# Autodesk Inventor assembly: 1_Base
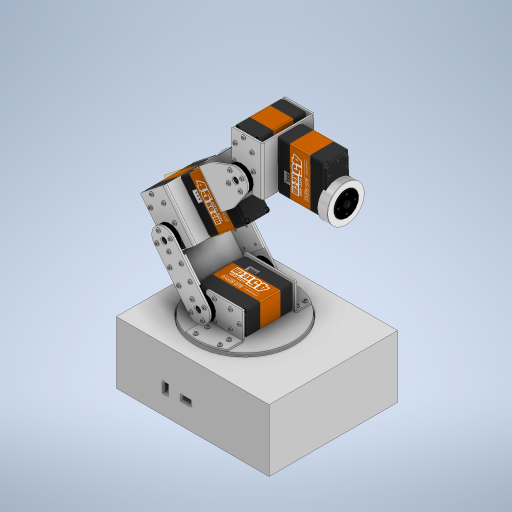
[picture p0: Inventor's stored thumbnail of the model, 512x512]
Saved by Autodesk Inventor 2024.2 (Build 282272000, 272)
## iProperties
Created: 2023-08-24
Part Number: 1_Base
Document SubType Name: Assembly
Designer: chanh
Author: chanh
## Documents named in this file (32)
- C:\Users\chanh\내 드라이브\로봇\Humanoid\Roboin Humanoid Project\Inventor\rh_plus_7_axis_robot_arm_hardware\Assembly\2_Arm.iam
- C:\Users\chanh\내 드라이브\로봇\Humanoid\Roboin Humanoid Project\Inventor\rh_plus_7_axis_robot_arm_hardware\Part\HTD-45H, Horn\HTD-45H\HTD-45H.ipt
- C:\Users\chanh\내 드라이브\로봇\Humanoid\Roboin Humanoid Project\Inventor\rh_plus_7_axis_robot_arm_hardware\Part\Frame\axis_1_top_frame.ipt
- C:\Users\chanh\내 드라이브\로봇\Humanoid\Roboin Humanoid Project\Inventor\rh_plus_7_axis_robot_arm_hardware\Part\Other Parts\Aluminum_Profile_4040_100.14mm_top.ipt
- C:\Users\chanh\내 드라이브\로봇\Humanoid\Roboin Humanoid Project\Inventor\rh_plus_7_axis_robot_arm_hardware\Part\Other Parts\Aluminum_Profile_4040_40.10mm_right.ipt
- C:\Users\chanh\내 드라이브\로봇\Humanoid\Roboin Humanoid Project\Inventor\rh_plus_7_axis_robot_arm_hardware\Part\Other Parts\Aluminum_Profile_4040_40.10mm_left.ipt
- C:\Users\chanh\내 드라이브\로봇\Humanoid\Roboin Humanoid Project\Inventor\rh_plus_7_axis_robot_arm_hardware\Part\Other Parts\Aluminum_Profile_4040_100.14mm_bottom.ipt
- C:\Users\chanh\내 드라이브\로봇\Humanoid\Roboin Humanoid Project\Inventor\rh_plus_7_axis_robot_arm_hardware\Part\HTD-45H, Horn\HTD-45H\M2x32.ipt
- C:\Users\chanh\내 드라이브\로봇\Humanoid\Roboin Humanoid Project\Inventor\rh_plus_7_axis_robot_arm_hardware\Part\HTD-45H, Horn\Horn\Top Horn.ipt
- C:\Users\chanh\내 드라이브\로봇\Humanoid\Roboin Humanoid Project\Inventor\rh_plus_7_axis_robot_arm_hardware\Part\Bolt, Bearing, Nut, Washer\M2x6 Round Bolt.ipt
- C:\Users\chanh\내 드라이브\로봇\Humanoid\Roboin Humanoid Project\Inventor\rh_plus_7_axis_robot_arm_hardware\Part\Bolt, Bearing, Nut, Washer\M2x35 Round Bolt.ipt
- C:\Users\chanh\내 드라이브\로봇\Humanoid\Roboin Humanoid Project\Inventor\rh_plus_7_axis_robot_arm_hardware\Part\Frame\axis_2_bottom_frame.ipt
- C:\Users\chanh\내 드라이브\로봇\Humanoid\Roboin Humanoid Project\Inventor\rh_plus_7_axis_robot_arm_hardware\Part\Bolt, Bearing, Nut, Washer\AXK5070+AS Bearing.ipt
- C:\Users\chanh\내 드라이브\로봇\Humanoid\Roboin Humanoid Project\Inventor\rh_plus_7_axis_robot_arm_hardware\Part\Bolt, Bearing, Nut, Washer\M2x6 Bolt.ipt
- C:\Users\chanh\내 드라이브\로봇\Humanoid\Roboin Humanoid Project\Inventor\rh_plus_7_axis_robot_arm_hardware\Part\HTD-45H, Horn\HTD-45H\HTD-45H.iam
- C:\Users\chanh\내 드라이브\로봇\Humanoid\Roboin Humanoid Project\Inventor\rh_plus_7_axis_robot_arm_hardware\Part\HTD-45H, Horn\Horn\M3x6.ipt
- C:\Users\chanh\내 드라이브\로봇\Humanoid\Roboin Humanoid Project\Inventor\rh_plus_7_axis_robot_arm_hardware\Part\Frame\axis_2_bottom_L_frame(top).ipt
- C:\Users\chanh\내 드라이브\로봇\Humanoid\Roboin Humanoid Project\Inventor\rh_plus_7_axis_robot_arm_hardware\Part\Frame\axis_2_bottom_L_frame(bottom).ipt
- C:\Users\chanh\내 드라이브\로봇\Humanoid\Roboin Humanoid Project\Inventor\rh_plus_7_axis_robot_arm_hardware\Part\HTD-45H, Horn\Horn\Bottom Horn.ipt
- C:\Users\chanh\내 드라이브\로봇\Humanoid\Roboin Humanoid Project\Inventor\rh_plus_7_axis_robot_arm_hardware\Part\Bolt, Bearing, Nut, Washer\M2x4 Round Bolt.ipt
- C:\Users\chanh\내 드라이브\로봇\Humanoid\Roboin Humanoid Project\Inventor\rh_plus_7_axis_robot_arm_hardware\Part\Frame\axis_3_bottom_frame(top).ipt
- C:\Users\chanh\내 드라이브\로봇\Humanoid\Roboin Humanoid Project\Inventor\rh_plus_7_axis_robot_arm_hardware\Part\Frame\axis_3_bottom_frame(bottom).ipt
- C:\Users\chanh\내 드라이브\로봇\Humanoid\Roboin Humanoid Project\Inventor\rh_plus_7_axis_robot_arm_hardware\Part\Frame\axis_3_bottom_frame(middle).ipt
- C:\Users\chanh\내 드라이브\로봇\Humanoid\Roboin Humanoid Project\Inventor\rh_plus_7_axis_robot_arm_hardware\Part\Frame\axis_3_top_frame.ipt
- C:\Users\chanh\내 드라이브\로봇\Humanoid\Roboin Humanoid Project\Inventor\rh_plus_7_axis_robot_arm_hardware\Part\Frame\axis_4_top_frame.ipt
- C:\Users\chanh\내 드라이브\로봇\Humanoid\Roboin Humanoid Project\Inventor\rh_plus_7_axis_robot_arm_hardware\Part\Frame\axis_5_bottom_frame.ipt
- C:\Users\chanh\내 드라이브\로봇\Humanoid\Roboin Humanoid Project\Inventor\rh_plus_7_axis_robot_arm_hardware\Part\Frame\axis_5_top_frame.ipt
- C:\Users\chanh\내 드라이브\로봇\Humanoid\Roboin Humanoid Project\Inventor\rh_plus_7_axis_robot_arm_hardware\Part\Bolt, Bearing, Nut, Washer\2030 Teflon Sheet.ipt
- C:\Users\chanh\내 드라이브\로봇\Humanoid\Roboin Humanoid Project\Inventor\rh_plus_7_axis_robot_arm_hardware\Part\Frame\axis_6_top_frame.ipt
- C:\Users\chanh\내 드라이브\로봇\Humanoid\Roboin Humanoid Project\Inventor\rh_plus_7_axis_robot_arm_hardware\Part\HTD-45H, Horn\Horn\M3x5.ipt
- C:\Users\chanh\내 드라이브\로봇\Humanoid\Roboin Humanoid Project\Inventor\rh_plus_7_axis_robot_arm_hardware\Part\Other Parts\Bottom_Cover.ipt
- C:\Users\chanh\내 드라이브\로봇\Humanoid\Roboin Humanoid Project\Inventor\rh_plus_7_axis_robot_arm_hardware\Part\Bolt, Bearing, Nut, Washer\M5x14.ipt
## Components (161 placed, 30 different names)
1. Aluminum_Profile_4040_100.14mm_top:1 — Flush:13, Flush:14, Mate:2, Mate:3, Flush:15, Flush:16, Mate:4, Flush:17, Flush:18, Mate:6
2. Aluminum_Profile_4040_40.10mm_right:1 — Mate:3, Flush:15, Flush:16
3. Aluminum_Profile_4040_40.10mm_left:1 — Mate:4, Flush:17, Flush:18, Mate:5, Flush:20
4. Aluminum_Profile_4040_100.14mm_bottom:1 — Flush:19, Mate:5, Flush:20, Mate:19, Flush:27
5. Bottom_Cover:1 — Mate:19, Mate:20, Flush:27
6. HTD-45H:1 — Rotational:1, Mate:1, Flush:1, Flush:2, Flush:12, Flush:13, Flush:14, Mate:2, Flush:19, Rigid:1, Rigid:2, Mate:7, Mate:8
7. axis_1_top_frame:1 — Flush:11, Flush:12, Mate:6, Mate:9, Mate:20, Rigid:160, Rigid:161, Rigid:162, Rigid:163, Rigid:164, Rigid:165, Rigid:166, Rigid:167, Rigid:168, Rigid:169, Rigid:170
8. HTD-45H:2 [sub-assembly] — Flush:21, Mate:11, Flush:23, Flush:24, Mate:13, Mate:17, Rotational:2, Rigid:114
9. axis_2_bottom_frame:1 — Rigid:10, Rigid:18, Rigid:19, Rigid:20, Rigid:21, Flush:21, Mate:11, Mate:14
10. axis_2_bottom_L_frame(top):1 — Flush:23, Flush:24, Mate:13, Mate:14, Rigid:23, Rigid:24, Rigid:25, Rigid:26, Rigid:27, Rigid:28, Rigid:29, Rigid:30, Rigid:31
11. axis_2_bottom_L_frame(bottom):1 — Mate:17, Rigid:32, Rigid:33, Rigid:34, Rigid:35, Rigid:36, Rigid:37, Rigid:38, Rigid:39, Rigid:40, Rigid:41, Rigid:42, Rigid:43
12. HTD-45H:3 [sub-assembly] — Rotational:3, Flush:25, Mate:18, Flush:26
13. axis_3_bottom_frame(top):1 — Rigid:44, Rigid:45, Rigid:48, Rigid:49, Rigid:50, Rigid:51, Rigid:52, Rigid:53, Rigid:54, Rigid:55, Rigid:56, Rigid:57, Rigid:58, Rigid:59, Rigid:60
14. axis_3_bottom_frame(middle):1 — Rigid:48, Rigid:104
15. axis_3_bottom_frame(bottom):1 — Rigid:61, Rigid:62, Rigid:63, Rigid:64, Rigid:65, Rigid:66, Rigid:67, Rigid:68, Rigid:69, Rigid:70, Rigid:71, Rigid:72, Rigid:102, Rigid:103, Rigid:104
16. axis_3_top_frame:1 — Flush:25, Mate:18, Flush:26, Rigid:74, Rigid:75, Rigid:76, Rigid:77, Rigid:78, Rigid:79, Rigid:80, Rigid:81, Rigid:82, Rigid:83, Rigid:84, Rigid:85, Rigid:86, Rigid:87, Rigid:88, Rigid:89, Rigid:90
17. HTD-45H:4 — Rigid:90, Rigid:91, Rigid:92, Rotational:4, Rigid:106
18. 2030 Teflon Sheet:1 — Rigid:107
19. axis_4_top_frame:1 — Rigid:106, Rigid:107, Rigid:155, Rigid:156, Rigid:157, Rigid:158
20. HTD-45H:5 [sub-assembly] — Rigid:105, Rotational:5
21. 2030 Teflon Sheet:2 — Rigid:108
22. axis_5_bottom_frame:1 — Rigid:99, Rigid:108, Rigid:126, Rigid:127, Rigid:128, Rigid:129, Rigid:130, Rigid:131, Rigid:132, Rigid:133, Rigid:134, Rigid:135, Rigid:136, Rigid:137, Rigid:138, Rigid:159
23. axis_5_top_frame:1 — Rigid:105, Rigid:111, Rigid:139, Rigid:140, Rigid:141, Rigid:142, Rigid:143, Rigid:144, Rigid:145, Rigid:146, Rigid:147, Rigid:148, Rigid:149, Rigid:150, Rigid:151, Rigid:152, Rigid:153, Rigid:154
24. HTD-45H:6 — Rigid:111, Rigid:112, Rotational:6
25. 2030 Teflon Sheet:3 — Rigid:125
26. axis_6_top_frame:1 — Rigid:112, Rigid:120, Rigid:121, Rigid:122, Rigid:123, Rigid:125
27. M2x32:1 — Rigid:2
28. M2x32:2 — Rigid:1
29. Top Horn:1 — Rotational:1, Rigid:10, Rigid:22
30. M5x14:1 — Rigid:160
31. M5x14:2 — Rigid:163
32. M5x14:3 — Rigid:161
33. M5x14:4 — Rigid:162
34. M3x6:1 — Rigid:22
35. M2x6 Round Bolt:3 — Rigid:168
36. M2x6 Round Bolt:4 — Rigid:170
37. M2x6 Round Bolt:5 — Rigid:169
38. AXK5070+AS Bearing:1 — Mate:7, Mate:8, Mate:9
39. M2x6 Round Bolt:1 — Rigid:167
40. M2x6 Round Bolt:2 — Rigid:166
41. M2x35 Round Bolt:1 — Rigid:165
42. M2x35 Round Bolt:2 — Rigid:164
43. Bottom Horn:5 — Rigid:102
44. Top Horn:2 — Rotational:2, Rigid:44, Rigid:113
45. M3x5:1 — Rigid:114
46. M3x6:2 — Rigid:113
47. M2x6 Bolt:1 — Rigid:18
48. M2x6 Bolt:2 — Rigid:19
49. M2x6 Bolt:3 — Rigid:20
50. M2x6 Bolt:4 — Rigid:21
51. M2x4 Round Bolt:1 — Rigid:23
52. M2x4 Round Bolt:2 — Rigid:24
53. M2x4 Round Bolt:3 — Rigid:25
54. M2x4 Round Bolt:4 — Rigid:26
55. M2x4 Round Bolt:5 — Rigid:27
56. M2x4 Round Bolt:6 — Rigid:28
57. M2x4 Round Bolt:7 — Rigid:29
58. M2x4 Round Bolt:8 — Rigid:30
59. M2x4 Round Bolt:9 — Rigid:31
60. M2x4 Round Bolt:10 — Rigid:32
61. M2x4 Round Bolt:11 — Rigid:33
62. M2x4 Round Bolt:12 — Rigid:34
63. M2x4 Round Bolt:13 — Rigid:35
64. M2x4 Round Bolt:14 — Rigid:36
65. M2x4 Round Bolt:15 — Rigid:37
66. M2x4 Round Bolt:16 — Rigid:38
67. M2x4 Round Bolt:17 — Rigid:39
68. M2x4 Round Bolt:18 — Rigid:40
69. M2x4 Round Bolt:19 — Rigid:41
70. M2x4 Round Bolt:20 — Rigid:42
71. M2x4 Round Bolt:21 — Rigid:43
72. Bottom Horn:4 — Rigid:103, Rigid:116
73. Top Horn:3 — Rotational:3, Rigid:45, Rigid:115
74. M3x5:2 — Rigid:116
75. M3x6:3 — Rigid:115
76. M2x4 Round Bolt:22 — Rigid:50
77. M2x4 Round Bolt:23 — Rigid:51
78. M2x4 Round Bolt:24 — Rigid:52
79. M2x4 Round Bolt:25 — Rigid:49
80. M2x4 Round Bolt:26 — Rigid:53
81. M2x4 Round Bolt:27 — Rigid:54
82. M2x4 Round Bolt:28 — Rigid:55
83. M2x4 Round Bolt:29 — Rigid:56
84. M2x4 Round Bolt:30 — Rigid:57
85. M2x4 Round Bolt:31 — Rigid:58
86. M2x4 Round Bolt:32 — Rigid:59
87. M2x4 Round Bolt:33 — Rigid:60
88. M2x4 Round Bolt:34 — Rigid:61
89. M2x4 Round Bolt:35 — Rigid:62
90. M2x4 Round Bolt:36 — Rigid:63
91. M2x4 Round Bolt:37 — Rigid:64
92. M2x4 Round Bolt:38 — Rigid:65
93. M2x4 Round Bolt:39 — Rigid:66
94. M2x4 Round Bolt:40 — Rigid:67
95. M2x4 Round Bolt:41 — Rigid:68
96. M2x4 Round Bolt:42 — Rigid:69
97. M2x4 Round Bolt:43 — Rigid:70
98. M2x4 Round Bolt:44 — Rigid:71
99. M2x4 Round Bolt:45 — Rigid:72
100. M2x4 Round Bolt:46 — Rigid:74
101. M2x4 Round Bolt:47 — Rigid:75
102. M2x4 Round Bolt:48 — Rigid:76
103. M2x4 Round Bolt:49 — Rigid:77
104. M2x4 Round Bolt:50 — Rigid:78
105. M2x4 Round Bolt:51 — Rigid:79
106. M2x4 Round Bolt:52 — Rigid:80
107. M2x4 Round Bolt:53 — Rigid:81
108. M2x4 Round Bolt:54 — Rigid:82
109. M2x4 Round Bolt:55 — Rigid:83
110. M2x4 Round Bolt:56 — Rigid:84
111. M2x4 Round Bolt:57 — Rigid:85
112. M2x4 Round Bolt:58 — Rigid:86
113. M2x4 Round Bolt:59 — Rigid:87
114. M2x4 Round Bolt:60 — Rigid:88
115. M2x4 Round Bolt:61 — Rigid:89
116. Top Horn:6 — Rotational:4, Rigid:99, Rigid:117
117. M3x6:4 — Rigid:117
118. M2x32:3 — Rigid:92
119. M2x32:4 — Rigid:91
120. M2x6 Round Bolt:6 — Rigid:155
121. M2x6 Round Bolt:7 — Rigid:156
122. M2x35 Round Bolt:3 — Rigid:157
123. M2x35 Round Bolt:4 — Rigid:158
124. Top Horn:7 — Rotational:5, Rigid:118, Rigid:159
125. Bottom Horn:3 — Rigid:119, Rigid:138
126. M3x6:5 — Rigid:118
127. M3x5:4 — Rigid:119
128. M2x4 Round Bolt:64 — Rigid:128
129. M2x4 Round Bolt:65 — Rigid:126
130. M2x4 Round Bolt:66 — Rigid:127
131. M2x4 Round Bolt:67 — Rigid:129
132. M2x4 Round Bolt:68 — Rigid:131
133. M2x4 Round Bolt:69 — Rigid:133
134. M2x4 Round Bolt:70 — Rigid:132
135. M2x4 Round Bolt:71 — Rigid:130
136. M2x4 Round Bolt:72 — Rigid:136
137. M2x4 Round Bolt:73 — Rigid:134
138. M2x4 Round Bolt:74 — Rigid:135
139. M2x4 Round Bolt:75 — Rigid:137
140. M2x4 Round Bolt:76 — Rigid:139
141. M2x4 Round Bolt:77 — Rigid:141
142. M2x4 Round Bolt:78 — Rigid:142
143. M2x4 Round Bolt:79 — Rigid:140
144. M2x4 Round Bolt:80 — Rigid:143
145. M2x4 Round Bolt:81 — Rigid:150
146. M2x4 Round Bolt:82 — Rigid:151
147. M2x4 Round Bolt:83 — Rigid:152
148. M2x4 Round Bolt:84 — Rigid:153
149. M2x4 Round Bolt:85 — Rigid:154
150. M2x4 Round Bolt:87 — Rigid:144
151. M2x4 Round Bolt:88 — Rigid:145
152. M2x4 Round Bolt:89 — Rigid:146
153. M2x4 Round Bolt:90 — Rigid:147
154. M2x4 Round Bolt:91 — Rigid:148
155. M2x4 Round Bolt:92 — Rigid:149
156. Top Horn:8 — Rotational:6, Rigid:124
157. M3x6:6 — Rigid:124
158. M2x4 Round Bolt:62 — Rigid:122
159. M2x4 Round Bolt:63 — Rigid:123
160. M2x35 Round Bolt:5 — Rigid:120
161. M2x35 Round Bolt:6 — Rigid:121
## Relationships (183: WeldJoint 143, Flush 18, Mate 16, RevoluteJoint 6)
- Rotational:1 [RevoluteJoint]: HTD-45H:1 ↔ Top Horn:1
- Rotational:2 [RevoluteJoint]: HTD-45H:2 ↔ Top Horn:2
- Rotational:3 [RevoluteJoint]: HTD-45H:3 ↔ Top Horn:3
- Rotational:4 [RevoluteJoint]: HTD-45H:4 ↔ Top Horn:6
- Rotational:5 [RevoluteJoint]: HTD-45H:5 ↔ Top Horn:7
- Rotational:6 [RevoluteJoint]: HTD-45H:6 ↔ Top Horn:8
- Mate:1: HTD-45H:1
- Flush:1: HTD-45H:1
- Flush:2: HTD-45H:1
- Flush:11: axis_1_top_frame:1
- Flush:12: HTD-45H:1 ↔ axis_1_top_frame:1
- Flush:13: Aluminum_Profile_4040_100.14mm_top:1 ↔ HTD-45H:1
- Flush:14: Aluminum_Profile_4040_100.14mm_top:1 ↔ HTD-45H:1
- Mate:2: Aluminum_Profile_4040_100.14mm_top:1 ↔ HTD-45H:1
- Mate:3: Aluminum_Profile_4040_100.14mm_top:1 ↔ Aluminum_Profile_4040_40.10mm_right:1
- Flush:15: Aluminum_Profile_4040_100.14mm_top:1 ↔ Aluminum_Profile_4040_40.10mm_right:1
- Flush:16: Aluminum_Profile_4040_100.14mm_top:1 ↔ Aluminum_Profile_4040_40.10mm_right:1
- Mate:4: Aluminum_Profile_4040_100.14mm_top:1 ↔ Aluminum_Profile_4040_40.10mm_left:1
- Flush:17: Aluminum_Profile_4040_100.14mm_top:1 ↔ Aluminum_Profile_4040_40.10mm_left:1
- Flush:18: Aluminum_Profile_4040_100.14mm_top:1 ↔ Aluminum_Profile_4040_40.10mm_left:1
- Flush:19: Aluminum_Profile_4040_100.14mm_bottom:1 ↔ HTD-45H:1
- Mate:5: Aluminum_Profile_4040_40.10mm_left:1 ↔ Aluminum_Profile_4040_100.14mm_bottom:1
- Flush:20: Aluminum_Profile_4040_40.10mm_left:1 ↔ Aluminum_Profile_4040_100.14mm_bottom:1
- Mate:6: Aluminum_Profile_4040_100.14mm_top:1 ↔ axis_1_top_frame:1
- Rigid:1 [WeldJoint]: HTD-45H:1 ↔ M2x32:2
- Rigid:2 [WeldJoint]: HTD-45H:1 ↔ M2x32:1
- Rigid:10 [WeldJoint]: axis_2_bottom_frame:1 ↔ Top Horn:1
- Mate:7: HTD-45H:1 ↔ AXK5070+AS Bearing:1
- Mate:8: HTD-45H:1 ↔ AXK5070+AS Bearing:1
- Mate:9: axis_1_top_frame:1 ↔ AXK5070+AS Bearing:1
- Rigid:18 [WeldJoint]: axis_2_bottom_frame:1 ↔ M2x6 Bolt:1
- Rigid:19 [WeldJoint]: axis_2_bottom_frame:1 ↔ M2x6 Bolt:2
- Rigid:20 [WeldJoint]: axis_2_bottom_frame:1 ↔ M2x6 Bolt:3
- Rigid:21 [WeldJoint]: axis_2_bottom_frame:1 ↔ M2x6 Bolt:4
- Rigid:22 [WeldJoint]: Top Horn:1 ↔ M3x6:1
- Flush:21: HTD-45H:2 ↔ axis_2_bottom_frame:1
- Mate:11: HTD-45H:2 ↔ axis_2_bottom_frame:1
- Flush:23: HTD-45H:2 ↔ axis_2_bottom_L_frame(top):1
- Flush:24 (-1 mm): HTD-45H:2 ↔ axis_2_bottom_L_frame(top):1
- Mate:13: HTD-45H:2 ↔ axis_2_bottom_L_frame(top):1
- Mate:14: axis_2_bottom_frame:1 ↔ axis_2_bottom_L_frame(top):1
- Mate:17: HTD-45H:2 ↔ axis_2_bottom_L_frame(bottom):1
- Rigid:23 [WeldJoint]: axis_2_bottom_L_frame(top):1 ↔ M2x4 Round Bolt:1
- Rigid:24 [WeldJoint]: axis_2_bottom_L_frame(top):1 ↔ M2x4 Round Bolt:2
- Rigid:25 [WeldJoint]: axis_2_bottom_L_frame(top):1 ↔ M2x4 Round Bolt:3
- Rigid:26 [WeldJoint]: axis_2_bottom_L_frame(top):1 ↔ M2x4 Round Bolt:4
- Rigid:27 [WeldJoint]: axis_2_bottom_L_frame(top):1 ↔ M2x4 Round Bolt:5
- Rigid:28 [WeldJoint]: axis_2_bottom_L_frame(top):1 ↔ M2x4 Round Bolt:6
- Rigid:29 [WeldJoint]: axis_2_bottom_L_frame(top):1 ↔ M2x4 Round Bolt:7
- Rigid:30 [WeldJoint]: axis_2_bottom_L_frame(top):1 ↔ M2x4 Round Bolt:8
- Rigid:31 [WeldJoint]: axis_2_bottom_L_frame(top):1 ↔ M2x4 Round Bolt:9
- Rigid:32 [WeldJoint]: axis_2_bottom_L_frame(bottom):1 ↔ M2x4 Round Bolt:10
- Rigid:33 [WeldJoint]: axis_2_bottom_L_frame(bottom):1 ↔ M2x4 Round Bolt:11
- Rigid:34 [WeldJoint]: axis_2_bottom_L_frame(bottom):1 ↔ M2x4 Round Bolt:12
- Rigid:35 [WeldJoint]: axis_2_bottom_L_frame(bottom):1 ↔ M2x4 Round Bolt:13
- Rigid:36 [WeldJoint]: axis_2_bottom_L_frame(bottom):1 ↔ M2x4 Round Bolt:14
- Rigid:37 [WeldJoint]: axis_2_bottom_L_frame(bottom):1 ↔ M2x4 Round Bolt:15
- Rigid:38 [WeldJoint]: axis_2_bottom_L_frame(bottom):1 ↔ M2x4 Round Bolt:16
- Rigid:39 [WeldJoint]: axis_2_bottom_L_frame(bottom):1 ↔ M2x4 Round Bolt:17
- Rigid:40 [WeldJoint]: axis_2_bottom_L_frame(bottom):1 ↔ M2x4 Round Bolt:18
- Rigid:41 [WeldJoint]: axis_2_bottom_L_frame(bottom):1 ↔ M2x4 Round Bolt:19
- Rigid:42 [WeldJoint]: axis_2_bottom_L_frame(bottom):1 ↔ M2x4 Round Bolt:20
- Rigid:43 [WeldJoint]: axis_2_bottom_L_frame(bottom):1 ↔ M2x4 Round Bolt:21
- Rigid:44 [WeldJoint]: axis_3_bottom_frame(top):1 ↔ Top Horn:2
- Rigid:45 [WeldJoint]: axis_3_bottom_frame(top):1 ↔ Top Horn:3
- Rigid:48 [WeldJoint]: axis_3_bottom_frame(top):1 ↔ axis_3_bottom_frame(middle):1
- Rigid:49 [WeldJoint]: axis_3_bottom_frame(top):1 ↔ M2x4 Round Bolt:25
- Rigid:50 [WeldJoint]: axis_3_bottom_frame(top):1 ↔ M2x4 Round Bolt:22
- Rigid:51 [WeldJoint]: axis_3_bottom_frame(top):1 ↔ M2x4 Round Bolt:23
- Rigid:52 [WeldJoint]: axis_3_bottom_frame(top):1 ↔ M2x4 Round Bolt:24
- Rigid:53 [WeldJoint]: axis_3_bottom_frame(top):1 ↔ M2x4 Round Bolt:26
- Rigid:54 [WeldJoint]: axis_3_bottom_frame(top):1 ↔ M2x4 Round Bolt:27
- Rigid:55 [WeldJoint]: axis_3_bottom_frame(top):1 ↔ M2x4 Round Bolt:28
- Rigid:56 [WeldJoint]: axis_3_bottom_frame(top):1 ↔ M2x4 Round Bolt:29
- Rigid:57 [WeldJoint]: axis_3_bottom_frame(top):1 ↔ M2x4 Round Bolt:30
- Rigid:58 [WeldJoint]: axis_3_bottom_frame(top):1 ↔ M2x4 Round Bolt:31
- Rigid:59 [WeldJoint]: axis_3_bottom_frame(top):1 ↔ M2x4 Round Bolt:32
- Rigid:60 [WeldJoint]: axis_3_bottom_frame(top):1 ↔ M2x4 Round Bolt:33
- Rigid:61 [WeldJoint]: axis_3_bottom_frame(bottom):1 ↔ M2x4 Round Bolt:34
- Rigid:62 [WeldJoint]: axis_3_bottom_frame(bottom):1 ↔ M2x4 Round Bolt:35
- Rigid:63 [WeldJoint]: axis_3_bottom_frame(bottom):1 ↔ M2x4 Round Bolt:36
- Rigid:64 [WeldJoint]: axis_3_bottom_frame(bottom):1 ↔ M2x4 Round Bolt:37
- Rigid:65 [WeldJoint]: axis_3_bottom_frame(bottom):1 ↔ M2x4 Round Bolt:38
- Rigid:66 [WeldJoint]: axis_3_bottom_frame(bottom):1 ↔ M2x4 Round Bolt:39
- Rigid:67 [WeldJoint]: axis_3_bottom_frame(bottom):1 ↔ M2x4 Round Bolt:40
- Rigid:68 [WeldJoint]: axis_3_bottom_frame(bottom):1 ↔ M2x4 Round Bolt:41
- Rigid:69 [WeldJoint]: axis_3_bottom_frame(bottom):1 ↔ M2x4 Round Bolt:42
- Rigid:70 [WeldJoint]: axis_3_bottom_frame(bottom):1 ↔ M2x4 Round Bolt:43
- Rigid:71 [WeldJoint]: axis_3_bottom_frame(bottom):1 ↔ M2x4 Round Bolt:44
- Rigid:72 [WeldJoint]: axis_3_bottom_frame(bottom):1 ↔ M2x4 Round Bolt:45
- Flush:25: HTD-45H:3 ↔ axis_3_top_frame:1
- Mate:18: HTD-45H:3 ↔ axis_3_top_frame:1
- Flush:26: HTD-45H:3 ↔ axis_3_top_frame:1
- Rigid:74 [WeldJoint]: axis_3_top_frame:1 ↔ M2x4 Round Bolt:46
- Rigid:75 [WeldJoint]: axis_3_top_frame:1 ↔ M2x4 Round Bolt:47
- Rigid:76 [WeldJoint]: axis_3_top_frame:1 ↔ M2x4 Round Bolt:48
- Rigid:77 [WeldJoint]: axis_3_top_frame:1 ↔ M2x4 Round Bolt:49
- Rigid:78 [WeldJoint]: axis_3_top_frame:1 ↔ M2x4 Round Bolt:50
- Rigid:79 [WeldJoint]: axis_3_top_frame:1 ↔ M2x4 Round Bolt:51
- Rigid:80 [WeldJoint]: axis_3_top_frame:1 ↔ M2x4 Round Bolt:52
- Rigid:81 [WeldJoint]: axis_3_top_frame:1 ↔ M2x4 Round Bolt:53
- Rigid:82 [WeldJoint]: axis_3_top_frame:1 ↔ M2x4 Round Bolt:54
- Rigid:83 [WeldJoint]: axis_3_top_frame:1 ↔ M2x4 Round Bolt:55
- Rigid:84 [WeldJoint]: axis_3_top_frame:1 ↔ M2x4 Round Bolt:56
- Rigid:85 [WeldJoint]: axis_3_top_frame:1 ↔ M2x4 Round Bolt:57
- Rigid:86 [WeldJoint]: axis_3_top_frame:1 ↔ M2x4 Round Bolt:58
- Rigid:87 [WeldJoint]: axis_3_top_frame:1 ↔ M2x4 Round Bolt:59
- Rigid:88 [WeldJoint]: axis_3_top_frame:1 ↔ M2x4 Round Bolt:60
- Rigid:89 [WeldJoint]: axis_3_top_frame:1 ↔ M2x4 Round Bolt:61
- Rigid:90 [WeldJoint]: axis_3_top_frame:1 ↔ HTD-45H:4
- Rigid:91 [WeldJoint]: HTD-45H:4 ↔ M2x32:4
- Rigid:92 [WeldJoint]: HTD-45H:4 ↔ M2x32:3
- Rigid:99 [WeldJoint]: axis_5_bottom_frame:1 ↔ Top Horn:6
- Rigid:102 [WeldJoint]: axis_3_bottom_frame(bottom):1 ↔ Bottom Horn:5
- Rigid:103 [WeldJoint]: axis_3_bottom_frame(bottom):1 ↔ Bottom Horn:4
- Rigid:104 [WeldJoint]: axis_3_bottom_frame(middle):1 ↔ axis_3_bottom_frame(bottom):1
- Rigid:105 [WeldJoint]: HTD-45H:5 ↔ axis_5_top_frame:1
- Rigid:106 [WeldJoint]: HTD-45H:4 ↔ axis_4_top_frame:1
- Rigid:107 [WeldJoint]: 2030 Teflon Sheet:1 ↔ axis_4_top_frame:1
- Rigid:108 [WeldJoint]: 2030 Teflon Sheet:2 ↔ axis_5_bottom_frame:1
- Rigid:111 [WeldJoint]: axis_5_top_frame:1 ↔ HTD-45H:6
- Rigid:112 [WeldJoint]: HTD-45H:6 ↔ axis_6_top_frame:1
- Rigid:113 [WeldJoint]: Top Horn:2 ↔ M3x6:2
- Rigid:114 [WeldJoint]: HTD-45H:2 ↔ M3x5:1
- Rigid:115 [WeldJoint]: Top Horn:3 ↔ M3x6:3
- Rigid:116 [WeldJoint]: Bottom Horn:4 ↔ M3x5:2
- Rigid:117 [WeldJoint]: Top Horn:6 ↔ M3x6:4
- Rigid:118 [WeldJoint]: Top Horn:7 ↔ M3x6:5
- Rigid:119 [WeldJoint]: Bottom Horn:3 ↔ M3x5:4
- Rigid:120 [WeldJoint]: axis_6_top_frame:1 ↔ M2x35 Round Bolt:5
- Rigid:121 [WeldJoint]: axis_6_top_frame:1 ↔ M2x35 Round Bolt:6
- Rigid:122 [WeldJoint]: axis_6_top_frame:1 ↔ M2x4 Round Bolt:62
- Rigid:123 [WeldJoint]: axis_6_top_frame:1 ↔ M2x4 Round Bolt:63
- Rigid:124 [WeldJoint]: Top Horn:8 ↔ M3x6:6
- Rigid:125 [WeldJoint]: 2030 Teflon Sheet:3 ↔ axis_6_top_frame:1
- Rigid:126 [WeldJoint]: axis_5_bottom_frame:1 ↔ M2x4 Round Bolt:65
- Rigid:127 [WeldJoint]: axis_5_bottom_frame:1 ↔ M2x4 Round Bolt:66
- Rigid:128 [WeldJoint]: axis_5_bottom_frame:1 ↔ M2x4 Round Bolt:64
- Rigid:129 [WeldJoint]: axis_5_bottom_frame:1 ↔ M2x4 Round Bolt:67
- Rigid:130 [WeldJoint]: axis_5_bottom_frame:1 ↔ M2x4 Round Bolt:71
- Rigid:131 [WeldJoint]: axis_5_bottom_frame:1 ↔ M2x4 Round Bolt:68
- Rigid:132 [WeldJoint]: axis_5_bottom_frame:1 ↔ M2x4 Round Bolt:70
- Rigid:133 [WeldJoint]: axis_5_bottom_frame:1 ↔ M2x4 Round Bolt:69
- Rigid:134 [WeldJoint]: axis_5_bottom_frame:1 ↔ M2x4 Round Bolt:73
- Rigid:135 [WeldJoint]: axis_5_bottom_frame:1 ↔ M2x4 Round Bolt:74
- Rigid:136 [WeldJoint]: axis_5_bottom_frame:1 ↔ M2x4 Round Bolt:72
- Rigid:137 [WeldJoint]: axis_5_bottom_frame:1 ↔ M2x4 Round Bolt:75
- Rigid:138 [WeldJoint]: axis_5_bottom_frame:1 ↔ Bottom Horn:3
- Rigid:139 [WeldJoint]: axis_5_top_frame:1 ↔ M2x4 Round Bolt:76
- Rigid:140 [WeldJoint]: axis_5_top_frame:1 ↔ M2x4 Round Bolt:79
- Rigid:141 [WeldJoint]: axis_5_top_frame:1 ↔ M2x4 Round Bolt:77
- Rigid:142 [WeldJoint]: axis_5_top_frame:1 ↔ M2x4 Round Bolt:78
- Rigid:143 [WeldJoint]: axis_5_top_frame:1 ↔ M2x4 Round Bolt:80
- Rigid:144 [WeldJoint]: axis_5_top_frame:1 ↔ M2x4 Round Bolt:87
- Rigid:145 [WeldJoint]: axis_5_top_frame:1 ↔ M2x4 Round Bolt:88
- Rigid:146 [WeldJoint]: axis_5_top_frame:1 ↔ M2x4 Round Bolt:89
- Rigid:147 [WeldJoint]: axis_5_top_frame:1 ↔ M2x4 Round Bolt:90
- Rigid:148 [WeldJoint]: axis_5_top_frame:1 ↔ M2x4 Round Bolt:91
- Rigid:149 [WeldJoint]: axis_5_top_frame:1 ↔ M2x4 Round Bolt:92
- Rigid:150 [WeldJoint]: axis_5_top_frame:1 ↔ M2x4 Round Bolt:81
- Rigid:151 [WeldJoint]: axis_5_top_frame:1 ↔ M2x4 Round Bolt:82
- Rigid:152 [WeldJoint]: axis_5_top_frame:1 ↔ M2x4 Round Bolt:83
- Rigid:153 [WeldJoint]: axis_5_top_frame:1 ↔ M2x4 Round Bolt:84
- Rigid:154 [WeldJoint]: axis_5_top_frame:1 ↔ M2x4 Round Bolt:85
- Rigid:155 [WeldJoint]: axis_4_top_frame:1 ↔ M2x6 Round Bolt:6
- Rigid:156 [WeldJoint]: axis_4_top_frame:1 ↔ M2x6 Round Bolt:7
- Rigid:157 [WeldJoint]: axis_4_top_frame:1 ↔ M2x35 Round Bolt:3
- Rigid:158 [WeldJoint]: axis_4_top_frame:1 ↔ M2x35 Round Bolt:4
- Rigid:159 [WeldJoint]: axis_5_bottom_frame:1 ↔ Top Horn:7
- Mate:19 (0.45 mm): Aluminum_Profile_4040_100.14mm_bottom:1 ↔ Bottom_Cover:1
- Mate:20 (0.5 mm): Bottom_Cover:1 ↔ axis_1_top_frame:1
- Flush:27: Aluminum_Profile_4040_100.14mm_bottom:1 ↔ Bottom_Cover:1
- Rigid:160 [WeldJoint]: axis_1_top_frame:1 ↔ M5x14:1
- Rigid:161 [WeldJoint]: axis_1_top_frame:1 ↔ M5x14:3
- Rigid:162 [WeldJoint]: axis_1_top_frame:1 ↔ M5x14:4
- Rigid:163 [WeldJoint]: axis_1_top_frame:1 ↔ M5x14:2
- Rigid:164 [WeldJoint]: axis_1_top_frame:1 ↔ M2x35 Round Bolt:2
- Rigid:165 [WeldJoint]: axis_1_top_frame:1 ↔ M2x35 Round Bolt:1
- Rigid:166 [WeldJoint]: axis_1_top_frame:1 ↔ M2x6 Round Bolt:2
- Rigid:167 [WeldJoint]: axis_1_top_frame:1 ↔ M2x6 Round Bolt:1
- Rigid:168 [WeldJoint]: axis_1_top_frame:1 ↔ M2x6 Round Bolt:3
- Rigid:169 [WeldJoint]: axis_1_top_frame:1 ↔ M2x6 Round Bolt:5
- Rigid:170 [WeldJoint]: axis_1_top_frame:1 ↔ M2x6 Round Bolt:4
